# Autodesk Inventor assembly: PivotAssembly_MIR
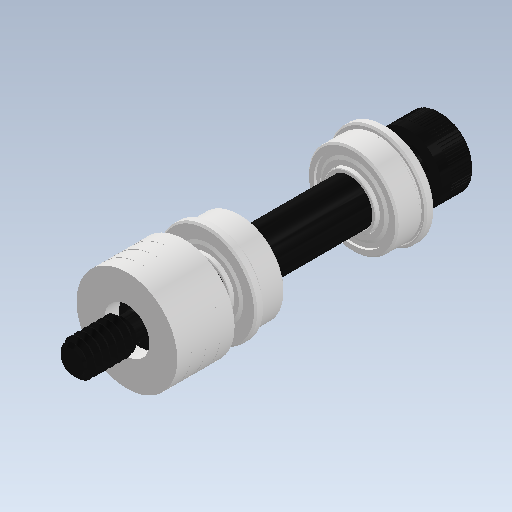
[picture p0: Inventor's stored thumbnail of the model, 512x512]
Saved by Autodesk Inventor 2023 (Build 270158000, 158)
## iProperties
Created: 2023-03-28
Part Number: PivotAssembly_MIR
Document SubType Name: Assembly
Designer: Dave
Author: Dave
## Documents named in this file (4)
- C:\Users\Dave\Documents\GitHub\BehrendURCMechanical\CAD\Chassis V3\Pivot Files and Assembly\PivotAssembly_MIR.iam
- C:\Users\Dave\Downloads\57155K337_Stainless Steel Ball Bearing_MIR.ipt
- C:\Users\Dave\Downloads\91259A546_Alloy Steel Shoulder Screw_MIR.ipt
- C:\Users\Dave\Downloads\96659A105_18-8 Stainless Steel SAE Washer_MIR.ipt
## Components (7 placed, 3 different names)
1. 57155K337_Stainless Steel Ball Bearing_MIR:1 — Mate:3, Mate:4, Mate:6
2. 91259A546_Alloy Steel Shoulder Screw_MIR:1 — Mate:3, Mate:8, Mate:2, Mate:1, Mate:5, Mate:10, Mate:12
3. 57155K337_Stainless Steel Ball Bearing_MIR:2 — Mate:4, Mate:2, Mate:1
4. 96659A105_18-8 Stainless Steel SAE Washer_MIR:1 — Mate:8, Mate:7, Mate:9
5. 96659A105_18-8 Stainless Steel SAE Washer_MIR:2 — Mate:7, Mate:6, Mate:5
6. 96659A105_18-8 Stainless Steel SAE Washer_MIR:3 — Mate:10, Mate:9, Mate:11
7. 96659A105_18-8 Stainless Steel SAE Washer_MIR:4 — Mate:12, Mate:11
## Relationships (12: Mate 12)
- Mate:3: 57155K337_Stainless Steel Ball Bearing_MIR:1 ↔ 91259A546_Alloy Steel Shoulder Screw_MIR:1
- Mate:8: 91259A546_Alloy Steel Shoulder Screw_MIR:1 ↔ 96659A105_18-8 Stainless Steel SAE Washer_MIR:1
- Mate:4 (-25.4 mm): 57155K337_Stainless Steel Ball Bearing_MIR:1 ↔ 57155K337_Stainless Steel Ball Bearing_MIR:2
- Mate:2 (3.175 mm): 91259A546_Alloy Steel Shoulder Screw_MIR:1 ↔ 57155K337_Stainless Steel Ball Bearing_MIR:2
- Mate:1: 91259A546_Alloy Steel Shoulder Screw_MIR:1 ↔ 57155K337_Stainless Steel Ball Bearing_MIR:2
- Mate:7: 96659A105_18-8 Stainless Steel SAE Washer_MIR:1 ↔ 96659A105_18-8 Stainless Steel SAE Washer_MIR:2
- Mate:6 (3.175 mm): 57155K337_Stainless Steel Ball Bearing_MIR:1 ↔ 96659A105_18-8 Stainless Steel SAE Washer_MIR:2
- Mate:5: 91259A546_Alloy Steel Shoulder Screw_MIR:1 ↔ 96659A105_18-8 Stainless Steel SAE Washer_MIR:2
- Mate:10: 91259A546_Alloy Steel Shoulder Screw_MIR:1 ↔ 96659A105_18-8 Stainless Steel SAE Washer_MIR:3
- Mate:9: 96659A105_18-8 Stainless Steel SAE Washer_MIR:1 ↔ 96659A105_18-8 Stainless Steel SAE Washer_MIR:3
- Mate:12: 91259A546_Alloy Steel Shoulder Screw_MIR:1 ↔ 96659A105_18-8 Stainless Steel SAE Washer_MIR:4
- Mate:11: 96659A105_18-8 Stainless Steel SAE Washer_MIR:3 ↔ 96659A105_18-8 Stainless Steel SAE Washer_MIR:4
